# Autodesk Inventor assembly: Chassis Assembly
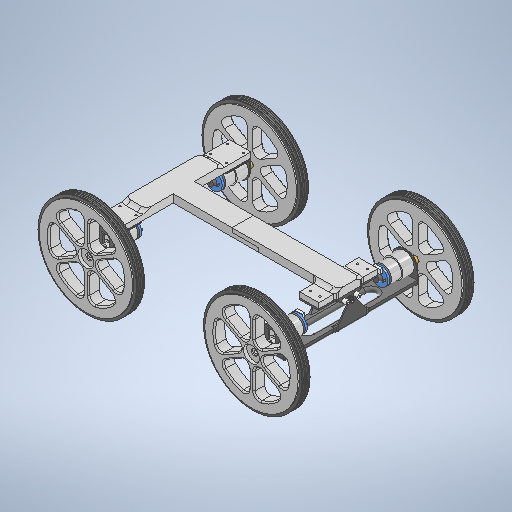
[picture p0: Inventor's stored thumbnail of the model, 512x512]
Saved by Autodesk Inventor 2025.2 (Build 292293000, 293)
## iProperties
Created: 2025-01-16
Part Number: Chassis Assembly
Document SubType Name: Assembly
Designer: Matt Tidd
Author: Matt Tidd
## Documents named in this file (5)
- C:\Users\mtidd2\Desktop\H2A\CAD\Chassis_Design\Chassis Assembly.iam
- C:\Users\mtidd2\Desktop\H2A\CAD\Motors_and_Wheels\Pendulum Suspension\Pendulum Suspension Assembly.iam
- C:\Users\mtidd2\Desktop\H2A\CAD\Motors_and_Wheels\Wheel Assembly\Motor Wheel Assembly.iam
- C:\Users\mtidd2\Desktop\H2A\CAD\Chassis_Design\Chassis Rear Spine.ipt
- C:\Users\mtidd2\Desktop\H2A\CAD\Chassis_Design\Chassis Front Spine.ipt
## Components (5 placed, 4 different names)
1. Motor Wheel Assembly:1 [sub-assembly] — Mate:1
2. Motor Wheel Assembly:2 [sub-assembly] — Mate:2
3. Pendulum Suspension Assembly:1 [sub-assembly] — Mate:3
4. Chassis Rear Spine:1 — Mate:1, Mate:2
5. Chassis Front Spine:1 — Mate:3
## Relationships (3: Mate 3)
- Mate:1: Motor Wheel Assembly:1 ↔ Chassis Rear Spine:1
- Mate:2: Motor Wheel Assembly:2 ↔ Chassis Rear Spine:1
- Mate:3: Pendulum Suspension Assembly:1 ↔ Chassis Front Spine:1
